# Autodesk Inventor assembly: FALCON GEARBOX2
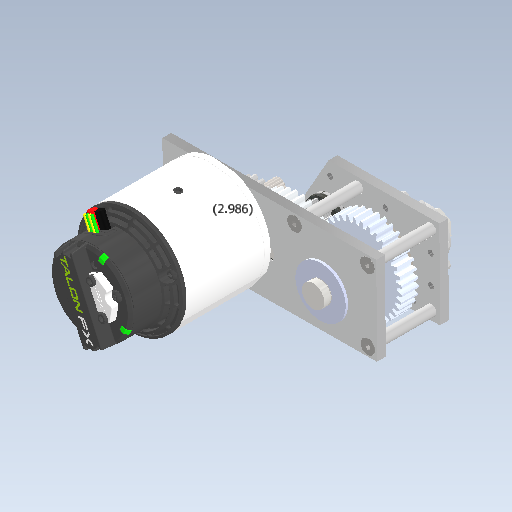
[picture p0: Inventor's stored thumbnail of the model, 512x512]
Saved by Autodesk Inventor 2021 (Build 250183000, 183)
## iProperties
Created: 2021-01-15
Part Number: FALCON GEARBOX2
Document SubType Name: Assembly
Designer: lucky
Mass: 857.274 g
Surface Area: 1196.01 cm^2
Volume: 256.441 cm^3
Density: 3.34296 g/cm^3
Author: lucky
## Documents named in this file (24)
- C:\Users\lucky\Documents\Inventor\2020DRIVEBASE\FALCON GEARBOX2.iam
- C:\Users\lucky\Documents\Inventor\2020DRIVEBASE\GEARBOX BACKPLATE.ipt
- C:\Users\lucky\Documents\Inventor\2020DRIVEBASE\GEARBOX FRONT PLATE.ipt
- C:\Users\lucky\Documents\Inventor\2020DRIVEBASE\0.5 Flanged Hex Bearing (1.125 OD) (217-3875).ipt
- C:\Users\lucky\Documents\Inventor\2020DRIVEBASE\AIS2020\W 619_8 R-2Z.iam
- C:\Users\lucky\Documents\Inventor\2020DRIVEBASE\Falcon 500, Powered by Talon FX (217-6515).ipt
- C:\Users\lucky\Documents\Inventor\2020DRIVEBASE\32T Aluminum Spur Gear (20 DP, 3_8_ Hex Bore) (217-5455).ipt
- C:\Users\lucky\Documents\Inventor\2020DRIVEBASE\36T Aluminum Spur Gear (20 DP, 1_2_ Hex Bore) (217-3214).ipt
- C:\Users\lucky\Documents\Inventor\2020DRIVEBASE\14T Aluminum Spur Gear (20 DP, 3_8_ Hex Bore) (217-2699).ipt
- C:\Users\lucky\Documents\Inventor\2020DRIVEBASE\14T Steel Spur Gear (20 DP, Falcon Motor) (217-6922).ipt
- C:\Users\lucky\Documents\Inventor\2020DRIVEBASE\PTO WEEK 4 TUESDAY\Workspace\WCP dual shifter\217-2731.ipt
- C:\Users\lucky\Documents\Inventor\2020DRIVEBASE\GEARBOX STANDOFFS.ipt
- C:\Users\lucky\Documents\Inventor\2020DRIVEBASE\Shaft6.ipt
- C:\Users\lucky\Documents\Inventor\2020DRIVEBASE\Shaft8.ipt
- C:\Users\lucky\Documents\Inventor\2020DRIVEBASE\FALCON GEARBOX2\Design Accelerator\Bolted Connection2.iam
- C:\Users\lucky\Documents\Inventor\2020DRIVEBASE\FALCON GEARBOX2\Design Accelerator\Bolted Connection3.iam
- C:\Users\lucky\Documents\Inventor\2020DRIVEBASE\FALCON GEARBOX2\Design Accelerator\Bolted Connection4.iam
- C:\Users\lucky\Documents\Inventor\2020DRIVEBASE\FALCON GEARBOX2\Design Accelerator\Bolted Connection5.iam
- C:\Users\lucky\Documents\Inventor\2020DRIVEBASE\FALCON GEARBOX2\Design Accelerator\Bolted Connection7.iam
- C:\Users\lucky\Documents\Inventor\2020DRIVEBASE\FALCON GEARBOX2\Design Accelerator\Bolted Connection8.iam
- C:\Users\lucky\Documents\Inventor\2020DRIVEBASE\FALCON GEARBOX2\Design Accelerator\Bolted Connection10.iam
- C:\Users\lucky\Documents\Inventor\2020DRIVEBASE\FALCON GEARBOX2\Design Accelerator\Bolted Connection11.iam
- C:\Users\lucky\Documents\Inventor\2020DRIVEBASE\12T Aluminum Hub Sprocket (#35 Chain, 1_2_ Hex Bore) (217-2662).ipt
- C:\Users\lucky\Documents\Inventor\2020DRIVEBASE\BEARINGSTANDIN.ipt
## Components (28 placed, 15 different names)
1. GEARBOX BACKPLATE:1 — Mate:1, Mate:2, Mate:6, Mate:8, Mate:11, Mate:12, Mate:13, Mate:14, Mate:24, Mate:25, Flush:1, Mate:26, Mate:28, Mate:29, Mate:30, Mate:31, Mate:48, Mate:49, Mate:50, Mate:51, Mate:52, Mate:53, Mate:54, Mate:55, Mate:62, Mate:64, Mate:70, Mate:71
2. GEARBOX FRONT PLATE:1 — Mate:1, Mate:4, Mate:7, Mate:9, Mate:13, Mate:27, Mate:32, Mate:38, Mate:39, Mate:40, Mate:41, Mate:42, Mate:43, Mate:44, Mate:45, Mate:65, Mate:66, Mate:69
3. 0.5 Flanged Hex Bearing (1.125 OD) (217-3875):1 — Mate:2, Mate:9, Mate:56, Angle:5
4. W 619_8 R-2Z:1 [sub-assembly] — Mate:4, Mate:7
5. W 619_8 R-2Z:2 [sub-assembly] — Mate:6, Mate:8, Mate:15, Mate:18, Mate:63
6. Falcon 500, Powered by Talon FX (217-6515):1 — Mate:11, Mate:12, Mate:16, Mate:17, Mate:70, Mate:71
7. 36T Aluminum Spur Gear (20 DP, 1_2_ Hex Bore) (217-3214):1 — Mate:14, Rotation:2, Angle:3, Flush:3
8. 32T Aluminum Spur Gear (20 DP, 3_8_ Hex Bore) (217-5455):1 — Mate:15, Mate:18, Mate:20, Rotation:1, Angle:1
9. 14T Aluminum Spur Gear (20 DP, 3_8_ Hex Bore) (217-2699):1 — Mate:20, Rotation:2, Angle:1, Angle:7, Mate:67, Mate:68, Flush:3
10. 14T Steel Spur Gear (20 DP, Falcon Motor) (217-6922):1 — Mate:16, Mate:17, Rotation:1
11. 217-2731:1 — Mate:24, Mate:25, Mate:57, Mate:58
12. GEARBOX STANDOFFS:1 — Flush:1, Mate:26
13. GEARBOX STANDOFFS:2 — Mate:27, Mate:28
14. GEARBOX STANDOFFS:3 — Mate:29, Mate:30
15. GEARBOX STANDOFFS:4 — Mate:31, Mate:32
16. Shaft:1 — Angle:3, Flush:2, Mate:57, Mate:58, Angle:5, Angle:6
17. Shaft:1 — Mate:63, Angle:7, Mate:64
18. Bolted Connection:1 [sub-assembly] — Mate:38, Mate:39
19. Bolted Connection:2 [sub-assembly] — Mate:40, Mate:41
20. Bolted Connection:3 [sub-assembly] — Mate:42, Mate:43
21. Bolted Connection:4 [sub-assembly] — Mate:44, Mate:45
22. Bolted Connection:6 [sub-assembly] — Mate:48, Mate:49
23. Bolted Connection:7 [sub-assembly] — Mate:50, Mate:51
24. Bolted Connection:8 [sub-assembly] — Mate:52, Mate:53
25. Bolted Connection:9 [sub-assembly] — Mate:54, Mate:55
26. 12T Aluminum Hub Sprocket (#35 Chain, 1_2_ Hex Bore) (217-2662):1 — Mate:56, Flush:2, Angle:6
27. BEARINGSTANDIN:1 — Mate:65, Mate:66, Mate:67, Mate:69
28. BEARINGSTANDIN:2 — Mate:62, Mate:68
## Relationships (64: Mate 54, Angle 5, Flush 3, RelateRotation 2)
- Mate:1: GEARBOX BACKPLATE:1 ↔ GEARBOX FRONT PLATE:1
- Mate:2: GEARBOX BACKPLATE:1 ↔ 0.5 Flanged Hex Bearing (1.125 OD) (217-3875):1
- Mate:4: GEARBOX FRONT PLATE:1 ↔ W 619_8 R-2Z:1
- Mate:6: GEARBOX BACKPLATE:1 ↔ W 619_8 R-2Z:2
- Mate:7: GEARBOX FRONT PLATE:1 ↔ W 619_8 R-2Z:1
- Mate:8: GEARBOX BACKPLATE:1 ↔ W 619_8 R-2Z:2
- Mate:9: GEARBOX FRONT PLATE:1 ↔ 0.5 Flanged Hex Bearing (1.125 OD) (217-3875):1
- Mate:11: GEARBOX BACKPLATE:1 ↔ Falcon 500, Powered by Talon FX (217-6515):1
- Mate:12: GEARBOX BACKPLATE:1 ↔ Falcon 500, Powered by Talon FX (217-6515):1
- Mate:13: GEARBOX BACKPLATE:1 ↔ GEARBOX FRONT PLATE:1
- Mate:14: GEARBOX BACKPLATE:1 ↔ 36T Aluminum Spur Gear (20 DP, 1_2_ Hex Bore) (217-3214):1
- Mate:15: W 619_8 R-2Z:2 ↔ 32T Aluminum Spur Gear (20 DP, 3_8_ Hex Bore) (217-5455):1
- Mate:16: Falcon 500, Powered by Talon FX (217-6515):1 ↔ 14T Steel Spur Gear (20 DP, Falcon Motor) (217-6922):1
- Mate:17: Falcon 500, Powered by Talon FX (217-6515):1 ↔ 14T Steel Spur Gear (20 DP, Falcon Motor) (217-6922):1
- Mate:18: W 619_8 R-2Z:2 ↔ 32T Aluminum Spur Gear (20 DP, 3_8_ Hex Bore) (217-5455):1
- Mate:20: 32T Aluminum Spur Gear (20 DP, 3_8_ Hex Bore) (217-5455):1 ↔ 14T Aluminum Spur Gear (20 DP, 3_8_ Hex Bore) (217-2699):1
- Rotation:1 [RelateRotation] (0.4375 ul): 32T Aluminum Spur Gear (20 DP, 3_8_ Hex Bore) (217-5455):1 ↔ 14T Steel Spur Gear (20 DP, Falcon Motor) (217-6922):1
- Rotation:2 [RelateRotation] (0.3889 ul): 36T Aluminum Spur Gear (20 DP, 1_2_ Hex Bore) (217-3214):1 ↔ 14T Aluminum Spur Gear (20 DP, 3_8_ Hex Bore) (217-2699):1
- Angle:1 (0 deg): 32T Aluminum Spur Gear (20 DP, 3_8_ Hex Bore) (217-5455):1 ↔ 14T Aluminum Spur Gear (20 DP, 3_8_ Hex Bore) (217-2699):1
- Mate:24: GEARBOX BACKPLATE:1 ↔ 217-2731:1
- Mate:25: GEARBOX BACKPLATE:1 ↔ 217-2731:1
- Flush:1: GEARBOX BACKPLATE:1 ↔ GEARBOX STANDOFFS:1
- Mate:26: GEARBOX BACKPLATE:1 ↔ GEARBOX STANDOFFS:1
- Mate:27: GEARBOX FRONT PLATE:1 ↔ GEARBOX STANDOFFS:2
- Mate:28: GEARBOX BACKPLATE:1 ↔ GEARBOX STANDOFFS:2
- Mate:29: GEARBOX BACKPLATE:1 ↔ GEARBOX STANDOFFS:3
- Mate:30: GEARBOX BACKPLATE:1 ↔ GEARBOX STANDOFFS:3
- Mate:31: GEARBOX BACKPLATE:1 ↔ GEARBOX STANDOFFS:4
- Mate:32: GEARBOX FRONT PLATE:1 ↔ GEARBOX STANDOFFS:4
- Angle:3 (0 deg): 36T Aluminum Spur Gear (20 DP, 1_2_ Hex Bore) (217-3214):1 ↔ Shaft:1
- Mate:38: GEARBOX FRONT PLATE:1 ↔ Bolted Connection:1
- Mate:39: GEARBOX FRONT PLATE:1 ↔ Bolted Connection:1
- Mate:40: GEARBOX FRONT PLATE:1 ↔ Bolted Connection:2
- Mate:41: GEARBOX FRONT PLATE:1 ↔ Bolted Connection:2
- Mate:42: GEARBOX FRONT PLATE:1 ↔ Bolted Connection:3
- Mate:43: GEARBOX FRONT PLATE:1 ↔ Bolted Connection:3
- Mate:44: GEARBOX FRONT PLATE:1 ↔ Bolted Connection:4
- Mate:45: GEARBOX FRONT PLATE:1 ↔ Bolted Connection:4
- Mate:48: GEARBOX BACKPLATE:1 ↔ Bolted Connection:6
- Mate:49: GEARBOX BACKPLATE:1 ↔ Bolted Connection:6
- Mate:50: GEARBOX BACKPLATE:1 ↔ Bolted Connection:7
- Mate:51: GEARBOX BACKPLATE:1 ↔ Bolted Connection:7
- Mate:52: GEARBOX BACKPLATE:1 ↔ Bolted Connection:8
- Mate:53: GEARBOX BACKPLATE:1 ↔ Bolted Connection:8
- Mate:54: GEARBOX BACKPLATE:1 ↔ Bolted Connection:9
- Mate:55: GEARBOX BACKPLATE:1 ↔ Bolted Connection:9
- Mate:56: 0.5 Flanged Hex Bearing (1.125 OD) (217-3875):1 ↔ 12T Aluminum Hub Sprocket (#35 Chain, 1_2_ Hex Bore) (217-2662):1
- Flush:2: Shaft:1 ↔ 12T Aluminum Hub Sprocket (#35 Chain, 1_2_ Hex Bore) (217-2662):1
- Mate:57: 217-2731:1 ↔ Shaft:1
- Mate:58: 217-2731:1 ↔ Shaft:1
- Angle:5 (0 deg): 0.5 Flanged Hex Bearing (1.125 OD) (217-3875):1 ↔ Shaft:1
- Angle:6 (0 deg): Shaft:1 ↔ 12T Aluminum Hub Sprocket (#35 Chain, 1_2_ Hex Bore) (217-2662):1
- Mate:62: GEARBOX BACKPLATE:1 ↔ BEARINGSTANDIN:2
- Mate:63: W 619_8 R-2Z:2 ↔ Shaft:1
- Angle:7 (0 deg): 14T Aluminum Spur Gear (20 DP, 3_8_ Hex Bore) (217-2699):1 ↔ Shaft:1
- Mate:64: GEARBOX BACKPLATE:1 ↔ Shaft:1
- Mate:65: GEARBOX FRONT PLATE:1 ↔ BEARINGSTANDIN:1
- Mate:66: GEARBOX FRONT PLATE:1 ↔ BEARINGSTANDIN:1
- Mate:67: 14T Aluminum Spur Gear (20 DP, 3_8_ Hex Bore) (217-2699):1 ↔ BEARINGSTANDIN:1
- Mate:68 (10.2 mm): 14T Aluminum Spur Gear (20 DP, 3_8_ Hex Bore) (217-2699):1 ↔ BEARINGSTANDIN:2
- Flush:3: 36T Aluminum Spur Gear (20 DP, 1_2_ Hex Bore) (217-3214):1 ↔ 14T Aluminum Spur Gear (20 DP, 3_8_ Hex Bore) (217-2699):1
- Mate:69: GEARBOX FRONT PLATE:1 ↔ BEARINGSTANDIN:1
- Mate:70: GEARBOX BACKPLATE:1 ↔ Falcon 500, Powered by Talon FX (217-6515):1
- Mate:71: GEARBOX BACKPLATE:1 ↔ Falcon 500, Powered by Talon FX (217-6515):1
